# Autodesk Inventor assembly: HUDSON-1-46 COMPLETO
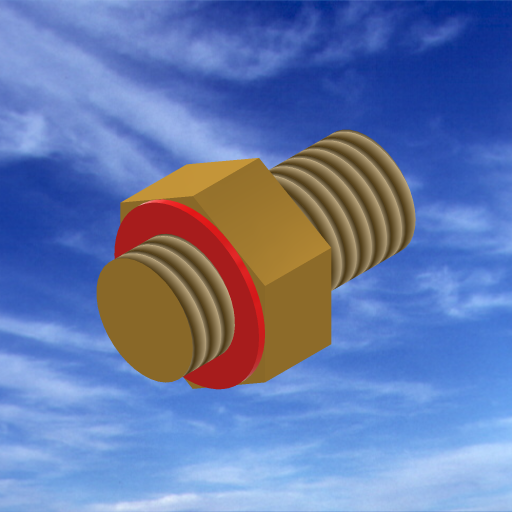
[picture p0: Inventor's stored thumbnail of the model, 512x512]
Saved by Autodesk Inventor 2024.2 (Build 282272000, 272)
## iProperties
Created: 2024-10-10
Part Number: HUDSON-1-46 COMPLETO
Document SubType Name: Assembly
Designer: Precisión-05
Author: Precisión-05
## Documents named in this file (3)
- C:\Users\Precisión-05\Desktop\LOCOMOTORA CABALLERO\HUDSON-1-46 COMPLETO.iam
- C:\Users\Precisión-05\Desktop\LOCOMOTORA CABALLERO\HUDSON-1-46-A.ipt
- C:\Users\Precisión-05\Desktop\LOCOMOTORA CABALLERO\Part8.ipt
## Components (2 placed, 2 different names)
1. HUDSON-1-46-A:1 — Rotational:1
2. Part8:1 — Rotational:1
## Relationships (1: RevoluteJoint 1)
- Rotational:1 [RevoluteJoint]: HUDSON-1-46-A:1 ↔ Part8:1
